# Autodesk Inventor assembly: Модуль_маркера
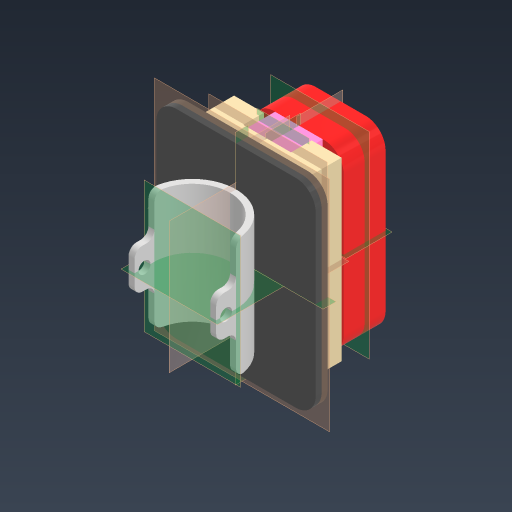
[picture p0: Inventor's stored thumbnail of the model, 512x512]
Saved by Autodesk Inventor 2023.2 (Build 272271030, 271C)
## iProperties
Created: 2026-01-03
Part Number: Модуль_маркера
Document SubType Name: Assembly
Designer: Олег Коноваленко
Author: Олег Коноваленко
## Documents named in this file (6)
- D:\VSOSH_IT_Robotics_ETZ\ETZ\Сonstruction\Модуль_маркера.iam
- D:\VSOSH_IT_Robotics_ETZ\ETZ\Сonstruction\Основание.ipt
- D:\VSOSH_IT_Robotics_ETZ\ETZ\Сonstruction\Направляющая.ipt
- D:\VSOSH_IT_Robotics_ETZ\ETZ\Сonstruction\Каретка.ipt
- D:\VSOSH_IT_Robotics_ETZ\ETZ\Сonstruction\Фанерка_маркера.ipt
- D:\VSOSH_IT_Robotics_ETZ\ETZ\Сonstruction\Крепление_маркера.ipt
## Components (5 placed, 5 different names)
1. Основание:1 — Совмещение:1, Совмещение:2, Заподлицо:1, Совмещение:3, Совмещение:4, Заподлицо:2
2. Направляющая:1 — Совмещение:3, Совмещение:4, Заподлицо:2, Совмещение:5, Совмещение:6
3. Каретка:1 — Совмещение:5, Совмещение:6, Совмещение:7, Совмещение:8, Совмещение:9
4. Фанерка_маркера:1 — Совмещение:7, Совмещение:8, Совмещение:9, Совмещение:10, Совмещение:11, Заподлицо:3
5. Крепление_маркера:1 — Совмещение:10, Совмещение:11, Заподлицо:3
## Relationships (14: Mate 11, Flush 3)
- Совмещение:1 [Mate]: Основание:1
- Совмещение:2 [Mate]: Основание:1
- Заподлицо:1 [Flush]: Основание:1
- Совмещение:3 [Mate]: Основание:1 ↔ Направляющая:1
- Совмещение:4 [Mate]: Основание:1 ↔ Направляющая:1
- Заподлицо:2 [Flush]: Основание:1 ↔ Направляющая:1
- Совмещение:5 [Mate]: Направляющая:1 ↔ Каретка:1
- Совмещение:6 [Mate]: Направляющая:1 ↔ Каретка:1
- Совмещение:7 [Mate]: Каретка:1 ↔ Фанерка_маркера:1
- Совмещение:8 [Mate]: Каретка:1 ↔ Фанерка_маркера:1
- Совмещение:9 [Mate]: Каретка:1 ↔ Фанерка_маркера:1
- Совмещение:10 [Mate]: Фанерка_маркера:1 ↔ Крепление_маркера:1
- Совмещение:11 [Mate] (12.5 mm): Фанерка_маркера:1 ↔ Крепление_маркера:1
- Заподлицо:3 [Flush]: Фанерка_маркера:1 ↔ Крепление_маркера:1
